# Autodesk Inventor assembly: OdometryWedgeBracket
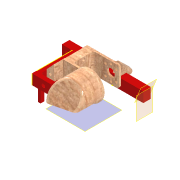
[picture p0: Inventor's stored thumbnail of the model, 180x180]
Saved by Autodesk Inventor 2020 (Build 240168000, 168)
## iProperties
Created: 2020-01-04
Part Number: OdometryWedgeBracket
Document SubType Name: Assembly
Designer: ball
Author: ball
## Documents named in this file (3)
- C:\FTC\FTC8863CAD\2019 Robot\Odoemetry module\OdometryWedgeBracket.iam
- C:\FTC\FTC8863CAD\2019 Robot\Odoemetry module\Odometry module wedge2-01.ipt
- C:\FTC\FTC8863CAD\2019 Robot\Odoemetry module\middleMountBracket.ipt
## Components (2 placed, 2 different names)
1. Odometry module wedge2-01:1 — Mate:1
2. middleMountBracket:1 — Mate:1
## Relationships (1: Mate 1)
- Mate:1: Odometry module wedge2-01:1 ↔ middleMountBracket:1
